# Autodesk Inventor assembly: Nema17_Schrittmotor
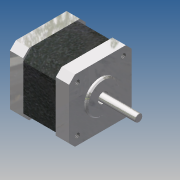
[picture p0: Inventor's stored thumbnail of the model, 180x180]
Saved by Autodesk Inventor 2015 (Build 190159000, 159)
## iProperties
Created: 2015-01-06
Part Number: Nema17_Schrittmotor
Document SubType Name: Assembly
Designer: Marc
Author: Marc
## Documents named in this file (5)
- E:\Modellflieger\3D Drucker\MotediusQR 400mm\Nema17 Schrittmotor\Nema17_Schrittmotor.iam
- E:\Modellflieger\3D Drucker\MotediusQR 400mm\Nema17 Schrittmotor\BackPlatte.ipt
- E:\Modellflieger\3D Drucker\MotediusQR 400mm\Nema17 Schrittmotor\Frontplatte.ipt
- E:\Modellflieger\3D Drucker\MotediusQR 400mm\Nema17 Schrittmotor\Mittelteil.ipt
- C:\Users\Marc\Documents\Inventor\Content Center Files\R2015\de-DE\DIN 84\DIN 84 - M4 x 8.ipt
## Components (7 placed, 4 different names)
1. BackPlatte:1 — Passend:1, Fluchtend:1, Fluchtend:2, Einfügen:1, Einfügen:2, Einfügen:3, Einfügen:4
2. Frontplatte:1 — Passend:2, Fluchtend:3, Fluchtend:4
3. Mittelteil:1 — Passend:1, Fluchtend:1, Fluchtend:2, Passend:2, Fluchtend:3, Fluchtend:4
4. DIN 84 - ersetzt durch DIN EN ISO 1207 M4 x 8:1 — Einfügen:1
5. DIN 84 - ersetzt durch DIN EN ISO 1207 M4 x 8:2 — Einfügen:2
6. DIN 84 - ersetzt durch DIN EN ISO 1207 M4 x 8:3 — Einfügen:3
7. DIN 84 - ersetzt durch DIN EN ISO 1207 M4 x 8:4 — Einfügen:4
## Relationships (10: Flush 4, Insert 4, Mate 2)
- Passend:1 [Mate]: BackPlatte:1 ↔ Mittelteil:1
- Fluchtend:1 [Flush]: BackPlatte:1 ↔ Mittelteil:1
- Fluchtend:2 [Flush]: BackPlatte:1 ↔ Mittelteil:1
- Passend:2 [Mate]: Frontplatte:1 ↔ Mittelteil:1
- Fluchtend:3 [Flush]: Frontplatte:1 ↔ Mittelteil:1
- Fluchtend:4 [Flush]: Frontplatte:1 ↔ Mittelteil:1
- Einfügen:1 [Insert]: BackPlatte:1 ↔ DIN 84 - ersetzt durch DIN EN ISO 1207 M4 x 8:1
- Einfügen:2 [Insert]: BackPlatte:1 ↔ DIN 84 - ersetzt durch DIN EN ISO 1207 M4 x 8:2
- Einfügen:3 [Insert]: BackPlatte:1 ↔ DIN 84 - ersetzt durch DIN EN ISO 1207 M4 x 8:3
- Einfügen:4 [Insert]: BackPlatte:1 ↔ DIN 84 - ersetzt durch DIN EN ISO 1207 M4 x 8:4
